# Autodesk Inventor assembly: arm
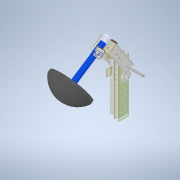
[picture p0: Inventor's stored thumbnail of the model, 180x180]
Saved by Autodesk Inventor 2021 (Build 250183000, 183)
## iProperties
Created: 2021-04-10
Part Number: arm
Document SubType Name: Assembly
Designer: gfellows
Author: gfellows
## Documents named in this file (18)
- C:\Users\gfellows\OneDrive - Eastside Preparatory School\Documents\arm.iam
- C:\Users\gfellows\Documents\GitHub\8103-CAD\1120-0010-0264.ipt
- C:\Users\gfellows\Documents\GitHub\8103-CAD\1603-0032-0012 assembly.ipt
- C:\Users\gfellows\Documents\GitHub\8103-CAD\525122.ipt
- C:\Users\gfellows\Documents\GitHub\8103-CAD\535118 assembly.ipt
- C:\Users\gfellows\Documents\GitHub\8103-CAD\545420.ipt
- C:\Users\gfellows\Documents\GitHub\8103-CAD\575112.ipt
- C:\Users\gfellows\Documents\GitHub\8103-CAD\DS3225-SG-Coreless.ipt
- C:\Users\gfellows\Documents\GitHub\8103-CAD\1201-0043-0002.ipt
- C:\Users\gfellows\Downloads\2302-0014-0060\2302-0014-0060.ipt
- C:\Users\gfellows\Downloads\1206-0016-0004\1206-0016-0004 assembly.ipt
- C:\Users\gfellows\Documents\GitHub\8103-CAD\2104 Series Aluminum REX Shaft (12mm Diameter, 240mm Length) 2104-0012-0240.ipt
- C:\Users\gfellows\Downloads\1301-0016-4012(1)\1301-0016-4012 assembly.ipt
- C:\Users\gfellows\Documents\GitHub\8103-CAD\1121-0006-0168.ipt
- C:\Users\gfellows\Downloads\1120-0002-0072.ipt
- C:\Users\gfellows\Downloads\am-4291 Wobble Goal.ipt
- C:\Users\gfellows\OneDrive - Eastside Preparatory School\Documents\grabber1.ipt
- C:\Users\gfellows\OneDrive - Eastside Preparatory School\Documents\grabber2.ipt
## Components (28 placed, 17 different names)
1. 1120-0010-0264:1 — Mate:1, Mate:18, Angle:7, Symmetry:2, Mate:20, Mate:21, Mate:22, Cylindrical:4, Angle:8, Angle:11, Cylindrical:5, Angle:12, Mate:39, Symmetry:3, Mate:46, Cylindrical:17, Angle:15
2. 1603-0032-0012 assembly:2 — Mate:20, Cylindrical:3, Cylindrical:4, Angle:8, Cylindrical:19
3. 1201-0043-0002:1 — Mate:21, Cylindrical:3, Mate:22, Symmetry:3
4. 1603-0032-0012 assembly:3 — Mate:46, Cylindrical:17, Angle:15
5. 525122:1 — Cylindrical:5, Mate:40, Cylindrical:10, Cylindrical:11
6. 535118 assembly:1 — Mate:36, Cylindrical:6, Angle:13, Cylindrical:7, Cylindrical:8, Mate:37, Mate:39
7. 545420:1 — Cylindrical:7, Cylindrical:8, Mate:37
8. 575112:1 — Angle:11, Mate:38, Cylindrical:9
9. 545420:2 — Mate:36, Cylindrical:6, Angle:13, Mate:38, Cylindrical:9
10. DS3225-SG-Coreless:1 — Angle:12
11. 2302-0014-0060:2 — Flush:27, Rotation:1, Cylindrical:15, Mate:48, Cylindrical:20
12. 1206-0016-0004 assembly:1 — Mate:40, Cylindrical:10, Cylindrical:11, Cylindrical:12, Cylindrical:13, Mate:41
13. 2302-0014-0060:3 — Cylindrical:12, Cylindrical:13, Mate:41, Flush:27, Rotation:1
14. 2104 Series Aluminum REX Shaft (12mm Diameter, 240mm Length) 2104-0012-0240:1 — Cylindrical:15, Mate:43, Mate:44, Angle:14, Cylindrical:18
15. 1301-0016-4012 assembly:1 — Mate:43, Mate:44, Flush:34
16. 1121-0006-0168:1 — Angle:14, Flush:30, Flush:31, Mate:48, Cylindrical:20, Cylindrical:21, Flush:35, Mate:49, Mate:64
17. 1121-0006-0168:2 — Flush:30, Flush:31, Mate:45, Cylindrical:18, Cylindrical:19, Flush:36, Mate:50, Flush:39
18. 1301-0016-4012 assembly:2 — Mate:45, Cylindrical:21, Flush:34
19. am-4291 Wobble Goal:1 — Flush:39
20. 1120-0002-0072:1 — Flush:35, Mate:49, Flush:36, Mate:50, Mate:63, Angle:66, Cylindrical:22, Flush:40, Flush:41
21. 525122:2 — Cylindrical:22
22. 535118 assembly:2 — Mate:63
23. 545420:3
24. 575112:2 — Angle:66
25. 545420:4 — Mate:64
26. DS3225-SG-Coreless:2
27. grabber1:1
28. grabber2:1 — Flush:40, Flush:41
## Relationships (80: Mate 38, CylindricalJoint 18, Angle 12, Flush 9, Symmetry 2, RelateRotation 1)
- Mate:1: 1120-0010-0264:1
- Mate:18: 1120-0010-0264:1
- Angle:7 (0 deg): 1120-0010-0264:1
- Symmetry:2: 1120-0010-0264:1
- Mate:19
- Mate:20: 1120-0010-0264:1 ↔ 1603-0032-0012 assembly:2
- Mate:21: 1120-0010-0264:1 ↔ 1201-0043-0002:1
- Cylindrical:3: 1603-0032-0012 assembly:2 ↔ 1201-0043-0002:1
- Mate:22: 1120-0010-0264:1 ↔ 1201-0043-0002:1
- Cylindrical:4: 1120-0010-0264:1 ↔ 1603-0032-0012 assembly:2
- Angle:8 (0 deg): 1120-0010-0264:1 ↔ 1603-0032-0012 assembly:2
- [Mate]: 575112:1 ↔ DS3225-SG-Coreless:1
- [Angle] (0 deg): 575112:1 ↔ DS3225-SG-Coreless:1
- [Mate]: 575112:1 ↔ 545420:2
- [Mate]: 525122:1 ↔ DS3225-SG-Coreless:1
- [Angle] (0 deg): 575112:1 ↔ 545420:2
- [Mate]: 525122:1 ↔ DS3225-SG-Coreless:1
- [Mate]: 575112:1 ↔ DS3225-SG-Coreless:1
- Angle:11 (0 deg): 1120-0010-0264:1 ↔ 575112:1
- Cylindrical:5: 1120-0010-0264:1 ↔ 525122:1
- Angle:12 (0 deg): 1120-0010-0264:1 ↔ DS3225-SG-Coreless:1
- Mate:36: 535118 assembly:1 ↔ 545420:2
- Cylindrical:6: 535118 assembly:1 ↔ 545420:2
- Angle:13 (0 deg): 535118 assembly:1 ↔ 545420:2
- Cylindrical:7: 535118 assembly:1 ↔ 545420:1
- Cylindrical:8: 535118 assembly:1 ↔ 545420:1
- Mate:37: 535118 assembly:1 ↔ 545420:1
- Mate:38: 575112:1 ↔ 545420:2
- Cylindrical:9: 575112:1 ↔ 545420:2
- Mate:39: 1120-0010-0264:1 ↔ 535118 assembly:1
- Mate:40: 525122:1 ↔ 1206-0016-0004 assembly:1
- Cylindrical:10: 525122:1 ↔ 1206-0016-0004 assembly:1
- Cylindrical:11: 525122:1 ↔ 1206-0016-0004 assembly:1
- Cylindrical:12: 1206-0016-0004 assembly:1 ↔ 2302-0014-0060:3
- Cylindrical:13: 1206-0016-0004 assembly:1 ↔ 2302-0014-0060:3
- Mate:41: 1206-0016-0004 assembly:1 ↔ 2302-0014-0060:3
- Flush:27: 2302-0014-0060:2 ↔ 2302-0014-0060:3
- Rotation:1 [RelateRotation] (1 ul): 2302-0014-0060:2 ↔ 2302-0014-0060:3
- Cylindrical:15: 2302-0014-0060:2 ↔ 2104 Series Aluminum REX Shaft (12mm Diameter, 240mm Length) 2104-0012-0240:1
- Mate:43: 2104 Series Aluminum REX Shaft (12mm Diameter, 240mm Length) 2104-0012-0240:1 ↔ 1301-0016-4012 assembly:1
- Mate:44: 2104 Series Aluminum REX Shaft (12mm Diameter, 240mm Length) 2104-0012-0240:1 ↔ 1301-0016-4012 assembly:1
- Symmetry:3: 1120-0010-0264:1 ↔ 1201-0043-0002:1
- Angle:14 (0 deg): 2104 Series Aluminum REX Shaft (12mm Diameter, 240mm Length) 2104-0012-0240:1 ↔ 1121-0006-0168:1
- Flush:30: 1121-0006-0168:1 ↔ 1121-0006-0168:2
- Flush:31: 1121-0006-0168:1 ↔ 1121-0006-0168:2
- Mate:45: 1121-0006-0168:2 ↔ 1301-0016-4012 assembly:2
- Mate:46: 1120-0010-0264:1 ↔ 1603-0032-0012 assembly:3
- Cylindrical:17: 1120-0010-0264:1 ↔ 1603-0032-0012 assembly:3
- Angle:15 (0 deg): 1120-0010-0264:1 ↔ 1603-0032-0012 assembly:3
- Mate:48: 2302-0014-0060:2 ↔ 1121-0006-0168:1
- Cylindrical:18: 2104 Series Aluminum REX Shaft (12mm Diameter, 240mm Length) 2104-0012-0240:1 ↔ 1121-0006-0168:2
- Cylindrical:19: 1603-0032-0012 assembly:2 ↔ 1121-0006-0168:2
- Cylindrical:20: 2302-0014-0060:2 ↔ 1121-0006-0168:1
- Cylindrical:21: 1121-0006-0168:1 ↔ 1301-0016-4012 assembly:2
- Flush:34: 1301-0016-4012 assembly:1 ↔ 1301-0016-4012 assembly:2
- Flush:35: 1121-0006-0168:1 ↔ 1120-0002-0072:1
- Mate:49: 1121-0006-0168:1 ↔ 1120-0002-0072:1
- Flush:36: 1121-0006-0168:2 ↔ 1120-0002-0072:1
- Mate:50: 1121-0006-0168:2 ↔ 1120-0002-0072:1
- [Mate]: 575112:2 ↔ DS3225-SG-Coreless:2
- [Angle] (0 deg): 575112:2 ↔ DS3225-SG-Coreless:2
- [Mate]: 575112:2 ↔ 545420:4
- [Mate]: 535118 assembly:2 ↔ 545420:4
- [Mate]: 535118 assembly:2 ↔ 545420:4
- [Mate]: 535118 assembly:2 ↔ 545420:4
- [Mate]: 535118 assembly:2 ↔ 545420:3
- [Mate]: 535118 assembly:2 ↔ 545420:3
- [Mate]: 535118 assembly:2 ↔ 545420:3
- [Mate]: 525122:2 ↔ DS3225-SG-Coreless:2
- [Mate]: 525122:2 ↔ 535118 assembly:2
- [Angle] (0 deg): 575112:2 ↔ 545420:4
- [Mate]: 525122:2 ↔ DS3225-SG-Coreless:2
- [Mate]: 575112:2 ↔ DS3225-SG-Coreless:2
- Mate:63: 1120-0002-0072:1 ↔ 535118 assembly:2
- Mate:64: 1121-0006-0168:1 ↔ 545420:4
- Angle:66 (0 deg): 1120-0002-0072:1 ↔ 575112:2
- Cylindrical:22: 1120-0002-0072:1 ↔ 525122:2
- Flush:39 (-6.35 mm): 1121-0006-0168:2 ↔ am-4291 Wobble Goal:1
- Flush:40: 1120-0002-0072:1 ↔ grabber2:1
- Flush:41: 1120-0002-0072:1 ↔ grabber2:1
## Named parameters: d159_d110 = 0 mm, d160_d94 = 0 mm, d161_d96 = 0 deg, d162_d97 = 0 mm, d163_d98 = 0 mm, d164_d99 = 0 mm, d165_d100 = 0 mm, d166_d101 = 0 mm, d167_d102 = 0 mm, d168_d103 = 0 mm, d169_d104 = 0 mm, d171_d106 = 0 deg, d172_d107 = 0 mm
